# Autodesk Inventor assembly: Pulley and Claw
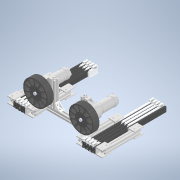
[picture p0: Inventor's stored thumbnail of the model, 180x180]
Saved by Autodesk Inventor 2020.2 (Build 242310000, 310)
## iProperties
Created: 2020-02-04
Part Number: Pulley and Claw
Document SubType Name: Assembly
Designer: AOFUser
Author: AOFUser
## Documents named in this file (6)
- C:\Users\AOFUser\Documents\GitHub\CAD\Robotics 2019-2020\Assembly\Pulley and Claw\Pulley and Claw.iam
- C:\Users\AOFUser\Documents\GitHub\CAD\Robotics 2019-2020\Assembly\Pulley and Claw\PulleySystem\PulleySystem Final.iam
- C:\Users\AOFUser\Documents\GitHub\CAD\Robotics 2019-2020\Assembly\Pulley and Claw\Claw\ClawAssembly.iam
- C:\Users\AOFUser\Documents\GitHub\CAD\Robotics 2019-2020\Assembly\Pulley and Claw\PulleySystem\1inchExtrusion.ipt
- C:\Users\AOFUser\Documents\GitHub\CAD\Robotics 2019-2020\Assembly\Pulley and Claw\Long Robotics Mount V2.ipt
- C:\Users\AOFUser\Documents\GitHub\CAD\Robotics 2019-2020\Assembly\PulleySystem\PulleySystem Final.iam
## Components (9 placed, 4 different names)
1. PulleySystem Final:1 [sub-assembly] — Rotational:1
2. ClawAssembly:1 [sub-assembly] — Mate:1, Flush:1, Mate:2, Flush:2
3. 1inchExtrusion:1 — Mate:1, Flush:1, Mate:3, Mate:4
4. 1inchExtrusion:2 — Mate:2, Flush:2, Mate:5, Mate:6
5. Long Robotics Mount V2:1 — Mate:3
6. Long Robotics Mount V2:2 — Mate:5, Rotational:2
7. Long Robotics Mount V2:3 — Mate:4, Rotational:1
8. Long Robotics Mount V2:4 — Mate:6
9. PulleySystem Final:2 [sub-assembly] — Rotational:2
## Relationships (10: Mate 6, Flush 2, RevoluteJoint 2)
- Mate:1: ClawAssembly:1 ↔ 1inchExtrusion:1
- Flush:1: ClawAssembly:1 ↔ 1inchExtrusion:1
- Mate:2: ClawAssembly:1 ↔ 1inchExtrusion:2
- Flush:2: ClawAssembly:1 ↔ 1inchExtrusion:2
- Mate:3: 1inchExtrusion:1 ↔ Long Robotics Mount V2:1
- Mate:4: 1inchExtrusion:1 ↔ Long Robotics Mount V2:3
- Rotational:1 [RevoluteJoint]: PulleySystem Final:1 ↔ Long Robotics Mount V2:3
- Mate:5: 1inchExtrusion:2 ↔ Long Robotics Mount V2:2
- Mate:6: 1inchExtrusion:2 ↔ Long Robotics Mount V2:4
- Rotational:2 [RevoluteJoint]: Long Robotics Mount V2:2 ↔ PulleySystem Final:2
